# Autodesk Inventor assembly: 30_Cube_Insert_Filter_Revolver_Filters_v3
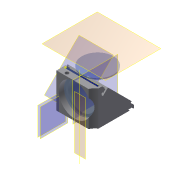
[picture p0: Inventor's stored thumbnail of the model, 180x180]
Saved by Autodesk Inventor 2019.4 (Build 234330000, 330)
## iProperties
Created: 2021-09-13
Part Number: 30_Cube_Insert_Filter_Revolver_Filters_v3
Document SubType Name: Assembly
Designer: diederichbenedict
Author: diederichbenedict
## Documents named in this file (5)
- C:\Users\diederichbenedict\Dropbox\Dokumente\Promotion\PROJECTS\UC2\02_CAD\INVENTOR\uc2_v3\30_Cube_Insert_Filter_Revolver_Filters_v3.iam
- C:\Users\diederichbenedict\Dropbox\Dokumente\Promotion\PROJECTS\UC2\02_CAD\INVENTOR\uc2_v3\00_Chroma_Dichroic_25x,3x1.ipt
- C:\Users\diederichbenedict\Dropbox\Dokumente\Promotion\PROJECTS\UC2\02_CAD\INVENTOR\uc2_v3\00_Comar_Filter_25Dia.ipt
- C:\Users\diederichbenedict\Dropbox\Dokumente\Promotion\PROJECTS\UC2\02_CAD\INVENTOR\uc2_v3\30_Cube_Insert_Filter_Revolver_Filter_base.ipt
- C:\Users\diederichbenedict\Dropbox\Dokumente\Promotion\PROJECTS\UC2\02_CAD\INVENTOR\uc2_v3\30_Cube_Insert_Filter_Revolver_Filter_clamp_v3.ipt
## Components (5 placed, 4 different names)
1. 00_Chroma_Dichroic_25x,3x1:1 — Mate:4, Mate:5
2. 00_Comar_Filter_25Dia:1
3. 30_Cube_Insert_Filter_Revolver_Filter_base:1
4. 00_Comar_Filter_25Dia:2 — Mate:4, Mate:5
5. 30_Cube_Insert_Filter_Revolver_Filter_clamp_v3:1
## Relationships (8: Mate 6, Flush 2)
- [Mate]: 00_Chroma_Dichroic_25x,3x1:1 ↔ 00_Comar_Filter_25Dia:1
- [Mate]: 00_Chroma_Dichroic_25x,3x1:1 ↔ 00_Comar_Filter_25Dia:1
- [Mate]: 00_Chroma_Dichroic_25x,3x1:1 ↔ 00_Comar_Filter_25Dia:1
- Mate:4: 00_Chroma_Dichroic_25x,3x1:1 ↔ 00_Comar_Filter_25Dia:2
- Mate:5: 00_Chroma_Dichroic_25x,3x1:1 ↔ 00_Comar_Filter_25Dia:2
- [Flush] (2 mm): 00_Chroma_Dichroic_25x,3x1:1 ↔ 30_Cube_Insert_Filter_Revolver_Filter_base:1
- [Mate]: 00_Chroma_Dichroic_25x,3x1:1 ↔ 30_Cube_Insert_Filter_Revolver_Filter_base:1
- [Flush]: 30_Cube_Insert_Filter_Revolver_Filter_base:1 ↔ 30_Cube_Insert_Filter_Revolver_Filter_clamp_v3:1
